# Autodesk Inventor assembly: knee
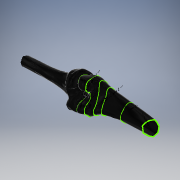
[picture p0: Inventor's stored thumbnail of the model, 180x180]
Saved by Autodesk Inventor 2019 (Build 230136000, 136)
## iProperties
Created: 2018-09-07
Part Number: knee
Document SubType Name: Assembly
Designer: HIVE
Author: HIVE
## Documents named in this file (2)
- E:\hive\projects\knee-patella\v4\knee.iam
- C:\Users\HIVE\Documents\Inventor\moment of inertia approximation reference.ipt
## Components (1 placed, 1 different names)
1. moment of inertia approximation reference:1 — Mate:1, Mate:2, Mate:3, Mate:4, Mate:5, Mate:6, Mate:7, Mate:8, Mate:9, Mate:10, Mate:11, Mate:12, Mate:13, Mate:14, Mate:15, Mate:16, Mate:17, Mate:18, Mate:19, Mate:20, Mate:21, Mate:22, Mate:23, Mate:24
## Relationships (24: Mate 24)
- Mate:1: moment of inertia approximation reference:1
- Mate:2: moment of inertia approximation reference:1
- Mate:3: moment of inertia approximation reference:1
- Mate:4: moment of inertia approximation reference:1
- Mate:5: moment of inertia approximation reference:1
- Mate:6: moment of inertia approximation reference:1
- Mate:7: moment of inertia approximation reference:1
- Mate:8: moment of inertia approximation reference:1
- Mate:9: moment of inertia approximation reference:1
- Mate:10: moment of inertia approximation reference:1
- Mate:11: moment of inertia approximation reference:1
- Mate:12: moment of inertia approximation reference:1
- Mate:13: moment of inertia approximation reference:1
- Mate:14: moment of inertia approximation reference:1
- Mate:15: moment of inertia approximation reference:1
- Mate:16: moment of inertia approximation reference:1
- Mate:17: moment of inertia approximation reference:1
- Mate:18: moment of inertia approximation reference:1
- Mate:19: moment of inertia approximation reference:1
- Mate:20: moment of inertia approximation reference:1
- Mate:21: moment of inertia approximation reference:1
- Mate:22: moment of inertia approximation reference:1
- Mate:23: moment of inertia approximation reference:1
- Mate:24: moment of inertia approximation reference:1
